# Autodesk Inventor assembly: Assembly1
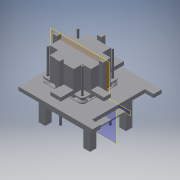
[picture p0: Inventor's stored thumbnail of the model, 180x180]
Saved by Autodesk Inventor 2019.3 (Build 233278000, 278)
## iProperties
Created: 2019-06-10
Part Number: Assembly1
Document SubType Name: Assembly
Designer: Frienddo
Author: Frienddo
## Documents named in this file (6)
- C:\Users\Frienddo\Desktop\HIVE-3Dprinters\Projects\Automate photogrametry\v3\control box\Assembly1.iam
- C:\Users\Frienddo\Desktop\HIVE-3Dprinters\Projects\Automate photogrametry\v3\control box\h bridge mount.ipt
- C:\Users\Frienddo\Desktop\HIVE-3Dprinters\Projects\Automate photogrametry\v3\control box\h bridge.ipt
- C:\Users\Frienddo\Desktop\HIVE-3Dprinters\Projects\Automate photogrametry\v3\control box\Protoboard mount.ipt
- C:\Users\Frienddo\Desktop\HIVE-3Dprinters\Projects\Automate photogrametry\v3\control box\Protoboard.ipt
- C:\Users\Frienddo\Desktop\HIVE-3Dprinters\Projects\Automate photogrametry\v3\control box\plate.ipt
## Components (5 placed, 5 different names)
1. h bridge mount:1 — Mate:1, Mate:2, Mate:5, Symmetry:1, Mate:8, Mate:10, Mate:11
2. h bridge:1 — Mate:2, Mate:5, Symmetry:1, Mate:8, Flush:1
3. Protoboard mount:1 — Mate:3, Mate:6, Flush:1, Flush:2, Mate:9, Flush:3
4. Protoboard:1 — Mate:3, Mate:6
5. plate:1 — Mate:9, Mate:10, Flush:3, Mate:11
## Relationships (13: Mate 9, Flush 3, Symmetry 1)
- Mate:1: h bridge mount:1
- Mate:2: h bridge mount:1 ↔ h bridge:1
- Mate:3: Protoboard mount:1 ↔ Protoboard:1
- Mate:5: h bridge mount:1 ↔ h bridge:1
- Mate:6: Protoboard mount:1 ↔ Protoboard:1
- Symmetry:1: h bridge mount:1 ↔ h bridge:1
- Mate:8: h bridge mount:1 ↔ h bridge:1
- Flush:1: h bridge:1 ↔ Protoboard mount:1
- Flush:2: Protoboard mount:1
- Mate:9: Protoboard mount:1 ↔ plate:1
- Mate:10: h bridge mount:1 ↔ plate:1
- Flush:3: Protoboard mount:1 ↔ plate:1
- Mate:11: h bridge mount:1 ↔ plate:1
